# Autodesk Inventor assembly: face
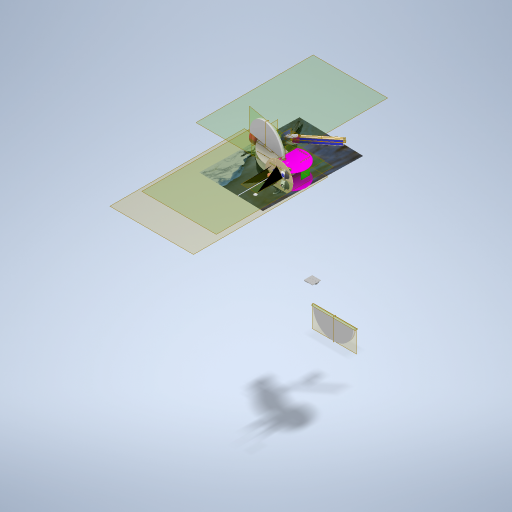
[picture p0: Inventor's stored thumbnail of the model, 512x512]
Saved by Autodesk Inventor 2023.2 (Build 272271030, 271C)
## iProperties
Created: 2024-01-26
Part Number: face
Document SubType Name: Assembly
Designer: I9232
Author: I9232
## Documents named in this file (48)
- D:\!project\fox_n_crow_construction\crow\face\face.iam
- D:\!project\fox_n_crow_construction\crow\face\Сборка глаза вороны.iam
- D:\!project\fox_n_crow_construction\crow\face\Деталь1.ipt
- D:\!project\fox_n_crow_construction\crow\face\Платформа для крыльев лево.ipt
- D:\!project\fox_n_crow_construction\crow\face\Платформа для крыльев право.ipt
- D:\!project\fox_n_crow_construction\crow\face\Сыр.ipt
- D:\!project\fox_n_crow_construction\crow\face\Веер.ipt
- D:\!project\fox_n_crow_construction\crow\face\боковые стороны головы.ipt
- D:\!project\fox_n_crow_construction\crow\face\servoDS3115mg.iam
- D:\!project\fox_n_crow_construction\crow\face\SERVO ARM HORN 25T ALUMINIUM\SERVO ARM HORN 25T ALUMINIUM.ipt
- D:\!project\fox_n_crow_construction\crow\face\Крепление рычага к лицу.ipt
- D:\!project\fox_n_crow_construction\crow\face\Лицо низ.ipt
- D:\!project\fox_n_crow_construction\crow\face\Лицо верх.ipt
- D:\!project\fox_n_crow_construction\crow\face\Шапка для головы вороны.ipt
- D:\!project\fox_n_crow_construction\crow\face\Крепление стрелялки.ipt
- D:\!project\fox_n_crow_construction\crow\cheese_shooter\Сборка стрелялки\Сборка стрелялки.iam
- D:\!project\fox_n_crow_construction\crow\face\клюв.ipt
- D:\!project\fox_n_crow_construction\crow\face\крепежная деталь для клюва.ipt
- D:\!project\fox_n_crow_construction\crow\face\Рычаг.ipt
- D:\!project\fox_n_crow_construction\crow\face\боковые стороны головы_MIR3.ipt
- D:\!project\fox_n_crow_construction\crow\face\Нижняя часть головы.ipt
- D:\!project\fox_n_crow_construction\crow\face\Деталь крепления механизма движения головы.ipt
- D:\!project\fox_n_crow_construction\crow\rotation_block\Povorot_mec.ipt.iam
- D:\!project\fox_n_crow_construction\crow\face\Деталь крепления механизма движения головы_MIR1.ipt
- D:\!project\fox_n_crow_construction\crow\face\Вал движения головы.ipt
- D:\!project\fox_n_crow_construction\crow\face\Крепление для крепления механизма головы.ipt
- D:\!project\fox_n_crow_construction\crow\rotation_block\User Library-Bearing KFL08.ipt
- D:\!project\fox_n_crow_construction\crow\face\Рычаг головы.ipt
- D:\!project\fox_n_crow_construction\crow\face\Шпилька.ipt
- D:\!project\fox_n_crow_construction\crow\face\Трубка.ipt
- D:\!project\fox_n_crow_construction\crow\rotation_block\SHF8_Горизонтальный_держатель_вала.ipt
- D:\!project\fox_n_crow_construction\crow\face\Фиксатор головы.ipt
- D:\!project\fox_n_crow_construction\crow\face\Вал фиксатора головы.ipt
- D:\!project\fox_n_crow_construction\crow\face\Нижняя часть головы_CPY.ipt
- D:\!project\fox_n_crow_construction\crow\face\Хвост.iam
- D:\!project\fox_n_crow_construction\crow\face\Петля.ipt
- D:\!project\fox_n_crow_construction\crow\face\Крепление хвоста.ipt
- D:\!project\fox_n_crow_construction\crow\face\Крепление хвоста(2 часть).ipt
- D:\!project\fox_n_crow_construction\crow\face\Ребро жёсткости для крепления хвоста.ipt
- D:\!project\fox_n_crow_construction\crow\face\Крепление хвоста(2 часть)_MIR2.ipt
- D:\!project\fox_n_crow_construction\crow\face\зрачок.ipt
- D:\!project\fox_n_crow_construction\crow\face\крыло.ipt
- D:\!project\fox_n_crow_construction\crow\face\Крыло(подвижная часть).ipt
- D:\!project\fox_n_crow_construction\crow\face\Ребро жётскости крыла.ipt
- D:\!project\fox_n_crow_construction\crow\face\Платформа для сервы в боковину.ipt
- D:\!project\fox_n_crow_construction\crow\face\Контур платы.ipt
- D:\!project\fox_n_crow_construction\crow\face\Фанерка ерпления колонок.ipt
- Povorot_mec.ipt
## Components (62 placed, 47 different names)
1. Сборка глаза вороны:1 [sub-assembly] — Заподлицо:1, Совмещение:39, Совмещение:129, Совмещение:145
2. Платформа глаз — Заподлицо:1, Заподлицо:4, Заподлицо:5, Заподлицо:6, Совмещение:27, Совмещение:28, Заподлицо:7, Заподлицо:8, Совмещение:39, Совмещение:53, Совмещение:80
3. Платформа для крыльев лево:1 — Совмещение:226, Совмещение:227, Совмещение:228
4. Сыр:1
5. Веер:1 — Совмещение:231, Совмещение:232, Совмещение:235
6. Веер:2
7. боковые стороны головы:1 — Совмещение:40, Совмещение:64, Совмещение:65, Заподлицо:10, Совмещение:81, Совмещение:97, Совмещение:116, Совмещение:169, Совмещение:172, Совмещение:173, Совмещение:179, Совмещение:180
8. servoDS3115mg:1 [sub-assembly] — Цилиндрический:10, Совмещение:40, Совмещение:43, Совмещение:64, Совмещение:65
9. Качалка сервы — Цилиндрический:10, Совмещение:43, Цилиндрический:21, Совмещение:168
10. Лицо низ:1 — Угол:2, Совмещение:54, Совмещение:56, Совмещение:57, Совмещение:109, Совмещение:150, Цилиндрический:24, Совмещение:185, Цилиндрический:25, Совмещение:189
11. Лицо верх:1 — Заподлицо:4, Заподлицо:5, Заподлицо:6, Угол:2, Совмещение:30, Совмещение:31, Совмещение:34, Совмещение:51, Совмещение:129, Цилиндрический:22, Цилиндрический:23, Совмещение:183, Совмещение:184, Совмещение:186, Совмещение:187
12. Шапка для головы вороны:1 — Совмещение:30
13. Крепление стрелялки:1 — Совмещение:27, Совмещение:28, Совмещение:32
14. Сборка стрелялки:1 [sub-assembly] — Заподлицо:7, Совмещение:31, Совмещение:32
15. клюв:2 — Совмещение:34, Заподлицо:8, Заподлицо:9, Совмещение:52
16. Крепление рычага к лицу:1 — Совмещение:56, Совмещение:57, Совмещение:109, Цилиндрический:20, Совмещение:182
17. крепежная деталь для клюва:1 — Совмещение:54, Совмещение:60
18. крепежная деталь для клюва:2 — Совмещение:51, Заподлицо:9, Совмещение:52
19. Рычаг:1 — Цилиндрический:20, Цилиндрический:21, Совмещение:168, Совмещение:182
20. клюв:3 — Совмещение:53, Совмещение:60, Совмещение:150, Совмещение:189
21. боковые стороны головы_MIR3:1 — Заподлицо:10, Совмещение:118, Совмещение:174, Совмещение:178, Совмещение:181
22. Нижняя часть головы:1 — Совмещение:179, Совмещение:180, Совмещение:181
23. Деталь крепления механизма движения головы:1 — Совмещение:151, Совмещение:154, Совмещение:157, Симметрия:1, Совмещение:164, Совмещение:165, Совмещение:167, Симметрия:2
24. Povorot_mec.ipt:1 [sub-assembly] — Совмещение:80, Совмещение:161, Совмещение:163
25. Деталь крепления механизма движения головы_MIR1:1 — Совмещение:152, Совмещение:156, Совмещение:158, Совмещение:159, Совмещение:160, Совмещение:161, Совмещение:162, Симметрия:1, Совмещение:166, Симметрия:2, Совмещение:190, Совмещение:205, Совмещение:212, Совмещение:233, Совмещение:234, Совмещение:239, Совмещение:240
26. Вал движения головы:1 — Совмещение:81, Совмещение:97, Совмещение:98, Совмещение:99, Совмещение:115, Совмещение:117, Совмещение:151, Совмещение:152
27. Ребро позвонок — Совмещение:145, Совмещение:167, Совмещение:201, Совмещение:203
28. Крепление рычага к лицу:2 — Цилиндрический:17, Совмещение:96
29. servoDS3115mg:2 [sub-assembly] — Цилиндрический:16, Совмещение:89, Совмещение:158, Совмещение:159, Совмещение:160
30. SERVO ARM HORN 25T ALUMINIUM:2 — Цилиндрический:16, Совмещение:89, Цилиндрический:18, Совмещение:128
31. User Library-Bearing KFL08:1 — Совмещение:99, Совмещение:108, Совмещение:139, Совмещение:141, Совмещение:142, Совмещение:144, Совмещение:154
32. Рычаг головы:1 — Цилиндрический:17, Цилиндрический:18, Совмещение:96, Совмещение:128
33. Шпилька:1 — Совмещение:104, Совмещение:133, Совмещение:141
34. User Library-Bearing KFL08:2 — Совмещение:98, Совмещение:104, Совмещение:105, Совмещение:140, Совмещение:162
35. Шпилька:2 — Совмещение:105, Совмещение:108, Совмещение:134, Совмещение:142
36. Трубка:1 — Совмещение:134, Совмещение:144, Совмещение:156, Совмещение:157
37. Трубка:2 — Совмещение:133, Совмещение:139, Совмещение:140
38. SHF8_Горизонтальный_держатель_вала:1 — Совмещение:115, Совмещение:116, Совмещение:169
39. SHF8_Горизонтальный_держатель_вала:2 — Совмещение:117, Совмещение:118, Совмещение:178
40. Фиксатор головы:1 — Цилиндрический:19, Совмещение:166
41. Вал фиксатора головы:1 — Цилиндрический:19, Совмещение:164, Совмещение:165
42. Нижняя часть головы_CPY:1 — Совмещение:172, Совмещение:173, Совмещение:174
43. Хвост:1 [sub-assembly] — Совмещение:188, Совмещение:192, Совмещение:198, Совмещение:199
44. Петля:1 — Цилиндрический:22, Совмещение:186, Совмещение:187, Цилиндрический:25
45. Петля:2 — Цилиндрический:23, Совмещение:183, Совмещение:184, Цилиндрический:24, Совмещение:185
46. Крепление хвоста:1 — Совмещение:190, Совмещение:200, Совмещение:203, Совмещение:204
47. Крепление хвоста(2 часть):1 — Совмещение:192, Совмещение:204
48. Ребро жёсткости для крепления хвоста:1 — Совмещение:200, Совмещение:201, Совмещение:202
49. Крепление хвоста(2 часть)_MIR2:1 — Совмещение:198, Совмещение:199
50. зрачок:1
51. зрачок:2
52. крыло:1 — Совмещение:205, Совмещение:213, Совмещение:214, Совмещение:217, Цилиндрический:26
53. Крыло(подвижная часть):1 — Совмещение:223, Совмещение:229, Совмещение:230
54. Петля:3 — Совмещение:217, Цилиндрический:26, Цилиндрический:27, Угол:3, Заподлицо:11
55. Ребро жётскости крыла:1 — Совмещение:212, Совмещение:213, Совмещение:214
56. Петля:4 — Цилиндрический:27, Угол:3, Заподлицо:11, Совмещение:223
57. servoDS3115mg:3 [sub-assembly] — Совмещение:226, Совмещение:227, Совмещение:228
58. Платформа для крыльев право:1 — Совмещение:229, Совмещение:230, Совмещение:231, Совмещение:232, Совмещение:235
59. Платформа для сервы в боковину:1 — Совмещение:233, Совмещение:234, Совмещение:236, Совмещение:237, Совмещение:238
60. servoDS3115mg:4 [sub-assembly] — Совмещение:236, Совмещение:237, Совмещение:238
61. Контур платы:1 — Совмещение:239
62. Фанерка ерпления колонок:1 — Совмещение:240
## Relationships (132: Mate 106, CylindricalJoint 13, Flush 9, Angle 2, Symmetry 2)
- Заподлицо:1 [Flush]: Сборка глаза вороны:1 ↔ Платформа глаз
- Заподлицо:4 [Flush]: Платформа глаз ↔ Лицо верх:1
- Заподлицо:5 [Flush]: Платформа глаз ↔ Лицо верх:1
- Заподлицо:6 [Flush]: Платформа глаз ↔ Лицо верх:1
- Угол:2 [Angle] (0 deg): Лицо низ:1 ↔ Лицо верх:1
- Совмещение:27 [Mate]: Платформа глаз ↔ Крепление стрелялки:1
- Совмещение:28 [Mate]: Платформа глаз ↔ Крепление стрелялки:1
- Совмещение:30 [Mate]: Лицо верх:1 ↔ Шапка для головы вороны:1
- Заподлицо:7 [Flush]: Платформа глаз ↔ Сборка стрелялки:1
- Совмещение:31 [Mate]: Лицо верх:1 ↔ Сборка стрелялки:1
- Совмещение:32 [Mate]: Крепление стрелялки:1 ↔ Сборка стрелялки:1
- Совмещение:34 [Mate]: Лицо верх:1 ↔ клюв:2
- Заподлицо:8 [Flush]: Платформа глаз ↔ клюв:2
- Совмещение:39 [Mate]: Сборка глаза вороны:1 ↔ Платформа глаз
- Цилиндрический:10 [CylindricalJoint]: servoDS3115mg:1 ↔ Качалка сервы
- Совмещение:40 [Mate]: боковые стороны головы:1 ↔ servoDS3115mg:1
- Совмещение:43 [Mate]: servoDS3115mg:1 ↔ Качалка сервы
- Совмещение:51 [Mate]: Лицо верх:1 ↔ крепежная деталь для клюва:2
- Заподлицо:9 [Flush]: клюв:2 ↔ крепежная деталь для клюва:2
- Совмещение:52 [Mate]: клюв:2 ↔ крепежная деталь для клюва:2
- Совмещение:53 [Mate]: Платформа глаз ↔ клюв:3
- Совмещение:54 [Mate]: Лицо низ:1 ↔ крепежная деталь для клюва:1
- Совмещение:56 [Mate]: Лицо низ:1 ↔ Крепление рычага к лицу:1
- Совмещение:57 [Mate]: Лицо низ:1 ↔ Крепление рычага к лицу:1
- Совмещение:60 [Mate]: крепежная деталь для клюва:1 ↔ клюв:3
- Совмещение:64 [Mate]: боковые стороны головы:1 ↔ servoDS3115mg:1
- Совмещение:65 [Mate]: боковые стороны головы:1 ↔ servoDS3115mg:1
- Заподлицо:10 [Flush]: боковые стороны головы:1 ↔ боковые стороны головы_MIR3:1
- Совмещение:80 [Mate]: Платформа глаз ↔ Povorot_mec.ipt:1
- Совмещение:81 [Mate]: боковые стороны головы:1 ↔ Вал движения головы:1
- Цилиндрический:16 [CylindricalJoint]: servoDS3115mg:2 ↔ SERVO ARM HORN 25T ALUMINIUM:2
- Совмещение:89 [Mate]: servoDS3115mg:2 ↔ SERVO ARM HORN 25T ALUMINIUM:2
- Цилиндрический:17 [CylindricalJoint]: Крепление рычага к лицу:2 ↔ Рычаг головы:1
- Цилиндрический:18 [CylindricalJoint]: SERVO ARM HORN 25T ALUMINIUM:2 ↔ Рычаг головы:1
- Совмещение:96 [Mate]: Крепление рычага к лицу:2 ↔ Рычаг головы:1
- Совмещение:97 [Mate]: боковые стороны головы:1 ↔ Вал движения головы:1
- Совмещение:98 [Mate]: Вал движения головы:1 ↔ User Library-Bearing KFL08:2
- Совмещение:99 [Mate]: Вал движения головы:1 ↔ User Library-Bearing KFL08:1
- Совмещение:104 [Mate]: Шпилька:1 ↔ User Library-Bearing KFL08:2
- Совмещение:105 [Mate]: User Library-Bearing KFL08:2 ↔ Шпилька:2
- Совмещение:108 [Mate]: User Library-Bearing KFL08:1 ↔ Шпилька:2
- Совмещение:109 [Mate]: Лицо низ:1 ↔ Крепление рычага к лицу:1
- Совмещение:115 [Mate]: Вал движения головы:1 ↔ SHF8_Горизонтальный_держатель_вала:1
- Совмещение:116 [Mate]: боковые стороны головы:1 ↔ SHF8_Горизонтальный_держатель_вала:1
- Совмещение:117 [Mate]: Вал движения головы:1 ↔ SHF8_Горизонтальный_держатель_вала:2
- Совмещение:118 [Mate]: боковые стороны головы_MIR3:1 ↔ SHF8_Горизонтальный_держатель_вала:2
- Цилиндрический:19 [CylindricalJoint]: Фиксатор головы:1 ↔ Вал фиксатора головы:1
- Совмещение:128 [Mate]: SERVO ARM HORN 25T ALUMINIUM:2 ↔ Рычаг головы:1
- Совмещение:129 [Mate]: Сборка глаза вороны:1 ↔ Лицо верх:1
- Совмещение:133 [Mate]: Шпилька:1 ↔ Трубка:2
- Совмещение:134 [Mate]: Шпилька:2 ↔ Трубка:1
- Совмещение:139 [Mate]: User Library-Bearing KFL08:1 ↔ Трубка:2
- Совмещение:140 [Mate]: User Library-Bearing KFL08:2 ↔ Трубка:2
- Совмещение:141 [Mate] (8.5 mm): User Library-Bearing KFL08:1 ↔ Шпилька:1
- Совмещение:142 [Mate] (8.5 mm): User Library-Bearing KFL08:1 ↔ Шпилька:2
- Совмещение:144 [Mate]: User Library-Bearing KFL08:1 ↔ Трубка:1
- Совмещение:145 [Mate]: Сборка глаза вороны:1 ↔ Ребро позвонок
- Совмещение:150 [Mate]: Лицо низ:1 ↔ клюв:3
- Совмещение:151 [Mate]: Деталь крепления механизма движения головы:1 ↔ Вал движения головы:1
- Совмещение:152 [Mate]: Деталь крепления механизма движения головы_MIR1:1 ↔ Вал движения головы:1
- Совмещение:154 [Mate]: Деталь крепления механизма движения головы:1 ↔ User Library-Bearing KFL08:1
- Совмещение:156 [Mate]: Деталь крепления механизма движения головы_MIR1:1 ↔ Трубка:1
- Совмещение:157 [Mate]: Деталь крепления механизма движения головы:1 ↔ Трубка:1
- Совмещение:158 [Mate]: Деталь крепления механизма движения головы_MIR1:1 ↔ servoDS3115mg:2
- Совмещение:159 [Mate]: Деталь крепления механизма движения головы_MIR1:1 ↔ servoDS3115mg:2
- Совмещение:160 [Mate] (-4 mm): Деталь крепления механизма движения головы_MIR1:1 ↔ servoDS3115mg:2
- Совмещение:161 [Mate]: Povorot_mec.ipt:1 ↔ Деталь крепления механизма движения головы_MIR1:1
- Совмещение:162 [Mate]: Деталь крепления механизма движения головы_MIR1:1 ↔ User Library-Bearing KFL08:2
- Симметрия:1 [Symmetry]: Деталь крепления механизма движения головы:1 ↔ Деталь крепления механизма движения головы_MIR1:1
- Совмещение:163 [Mate]: Povorot_mec.ipt:1
- Совмещение:164 [Mate]: Деталь крепления механизма движения головы:1 ↔ Вал фиксатора головы:1
- Совмещение:165 [Mate]: Деталь крепления механизма движения головы:1 ↔ Вал фиксатора головы:1
- Совмещение:166 [Mate] (1 mm): Деталь крепления механизма движения головы_MIR1:1 ↔ Фиксатор головы:1
- Совмещение:167 [Mate]: Деталь крепления механизма движения головы:1 ↔ Ребро позвонок
- Цилиндрический:20 [CylindricalJoint]: Крепление рычага к лицу:1 ↔ Рычаг:1
- Цилиндрический:21 [CylindricalJoint]: Качалка сервы ↔ Рычаг:1
- Совмещение:168 [Mate]: Качалка сервы ↔ Рычаг:1
- Совмещение:169 [Mate]: боковые стороны головы:1 ↔ SHF8_Горизонтальный_держатель_вала:1
- Совмещение:172 [Mate]: боковые стороны головы:1 ↔ Нижняя часть головы_CPY:1
- Совмещение:173 [Mate]: боковые стороны головы:1 ↔ Нижняя часть головы_CPY:1
- Совмещение:174 [Mate]: боковые стороны головы_MIR3:1 ↔ Нижняя часть головы_CPY:1
- Совмещение:178 [Mate]: боковые стороны головы_MIR3:1 ↔ SHF8_Горизонтальный_держатель_вала:2
- Совмещение:179 [Mate]: боковые стороны головы:1 ↔ Нижняя часть головы:1
- Совмещение:180 [Mate]: боковые стороны головы:1 ↔ Нижняя часть головы:1
- Совмещение:181 [Mate]: боковые стороны головы_MIR3:1 ↔ Нижняя часть головы:1
- Совмещение:182 [Mate]: Крепление рычага к лицу:1 ↔ Рычаг:1
- Цилиндрический:22 [CylindricalJoint]: Лицо верх:1 ↔ Петля:1
- Цилиндрический:23 [CylindricalJoint]: Лицо верх:1 ↔ Петля:2
- Совмещение:183 [Mate]: Лицо верх:1 ↔ Петля:2
- Совмещение:184 [Mate]: Лицо верх:1 ↔ Петля:2
- Цилиндрический:24 [CylindricalJoint]: Лицо низ:1 ↔ Петля:2
- Совмещение:185 [Mate]: Лицо низ:1 ↔ Петля:2
- Совмещение:186 [Mate]: Лицо верх:1 ↔ Петля:1
- Совмещение:187 [Mate]: Лицо верх:1 ↔ Петля:1
- Цилиндрический:25 [CylindricalJoint]: Лицо низ:1 ↔ Петля:1
- Симметрия:2 [Symmetry]: Деталь крепления механизма движения головы:1 ↔ Деталь крепления механизма движения головы_MIR1:1
- Совмещение:188 [Mate]: Хвост:1
- Совмещение:189 [Mate]: Лицо низ:1 ↔ клюв:3
- Совмещение:190 [Mate]: Деталь крепления механизма движения головы_MIR1:1 ↔ Крепление хвоста:1
- Совмещение:192 [Mate]: Хвост:1 ↔ Крепление хвоста(2 часть):1
- Совмещение:198 [Mate]: Хвост:1 ↔ Крепление хвоста(2 часть)_MIR2:1
- Совмещение:199 [Mate]: Хвост:1 ↔ Крепление хвоста(2 часть)_MIR2:1
- Совмещение:200 [Mate]: Крепление хвоста:1 ↔ Ребро жёсткости для крепления хвоста:1
- Совмещение:201 [Mate]: Ребро позвонок ↔ Ребро жёсткости для крепления хвоста:1
- Совмещение:202 [Mate]: Ребро жёсткости для крепления хвоста:1
- Совмещение:203 [Mate]: Ребро позвонок ↔ Крепление хвоста:1
- Совмещение:204 [Mate]: Крепление хвоста:1 ↔ Крепление хвоста(2 часть):1
- Совмещение:205 [Mate]: Деталь крепления механизма движения головы_MIR1:1 ↔ крыло:1
- Совмещение:212 [Mate]: Деталь крепления механизма движения головы_MIR1:1 ↔ Ребро жётскости крыла:1
- Совмещение:213 [Mate]: крыло:1 ↔ Ребро жётскости крыла:1
- Совмещение:214 [Mate]: крыло:1 ↔ Ребро жётскости крыла:1
- Совмещение:217 [Mate]: крыло:1 ↔ Петля:3
- Цилиндрический:26 [CylindricalJoint]: крыло:1 ↔ Петля:3
- Цилиндрический:27 [CylindricalJoint]: Петля:3 ↔ Петля:4
- Угол:3 [Angle] (90 deg): Петля:3 ↔ Петля:4
- Заподлицо:11 [Flush]: Петля:3 ↔ Петля:4
- Совмещение:223 [Mate]: Крыло(подвижная часть):1 ↔ Петля:4
- Совмещение:226 [Mate]: Платформа для крыльев лево:1 ↔ servoDS3115mg:3
- Совмещение:227 [Mate]: Платформа для крыльев лево:1 ↔ servoDS3115mg:3
- Совмещение:228 [Mate]: Платформа для крыльев лево:1 ↔ servoDS3115mg:3
- Совмещение:229 [Mate]: Крыло(подвижная часть):1 ↔ Платформа для крыльев право:1
- Совмещение:230 [Mate]: Крыло(подвижная часть):1 ↔ Платформа для крыльев право:1
- Совмещение:231 [Mate]: Веер:1 ↔ Платформа для крыльев право:1
- Совмещение:232 [Mate]: Веер:1 ↔ Платформа для крыльев право:1
- Совмещение:233 [Mate]: Деталь крепления механизма движения головы_MIR1:1 ↔ Платформа для сервы в боковину:1
- Совмещение:234 [Mate]: Деталь крепления механизма движения головы_MIR1:1 ↔ Платформа для сервы в боковину:1
- Совмещение:235 [Mate]: Веер:1 ↔ Платформа для крыльев право:1
- Совмещение:236 [Mate]: Платформа для сервы в боковину:1 ↔ servoDS3115mg:4
- Совмещение:237 [Mate]: Платформа для сервы в боковину:1 ↔ servoDS3115mg:4
- Совмещение:238 [Mate]: Платформа для сервы в боковину:1 ↔ servoDS3115mg:4
- Совмещение:239 [Mate]: Деталь крепления механизма движения головы_MIR1:1 ↔ Контур платы:1
- Совмещение:240 [Mate]: Деталь крепления механизма движения головы_MIR1:1 ↔ Фанерка ерпления колонок:1
